# Autodesk Inventor assembly: BaugruppeM3
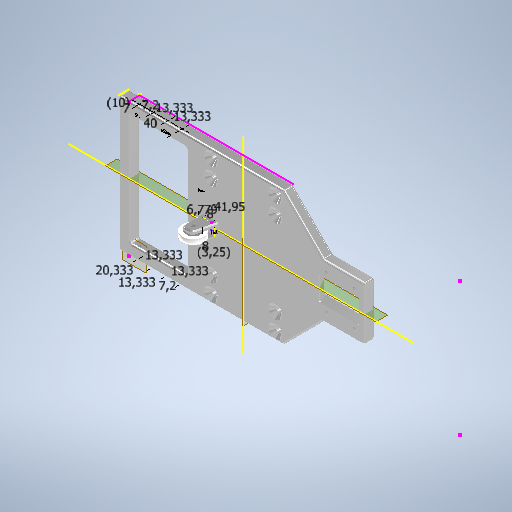
[picture p0: Inventor's stored thumbnail of the model, 512x512]
Saved by Autodesk Inventor 2025 (Build 290162010, 162A)
## iProperties
Created: 2025-01-24
Part Number: BaugruppeM3
Document SubType Name: Assembly
Designer: Admin
Author: Admin
## Documents named in this file (3)
- C:\Users\Admin\GIT\HDVKBM\CAD\Krandemonstrator\BaugruppeM3.iam
- C:\Users\Admin\GIT\HDVKBM\CAD\Krandemonstrator\SchlittenS.ipt
- C:\Users\Admin\GIT\HDVKBM\CAD\Krandemonstrator\UmlenkrolleHalterHeavy.iam
## Components (2 placed, 2 different names)
1. SchlittenS:1 — Verschiebbar:1, Planar:1
2. UmlenkrolleHalterHeavy:1 [sub-assembly] — Verschiebbar:1, Planar:1
## Relationships (2: TranslationJoint 1, PlanarJoint 1)
- Verschiebbar:1 [TranslationJoint]: SchlittenS:1 ↔ UmlenkrolleHalterHeavy:1
- Planar:1 (68.496 mm): SchlittenS:1 ↔ UmlenkrolleHalterHeavy:1
